# Autodesk Inventor assembly: 21-091-PHANTOM-HRDSET
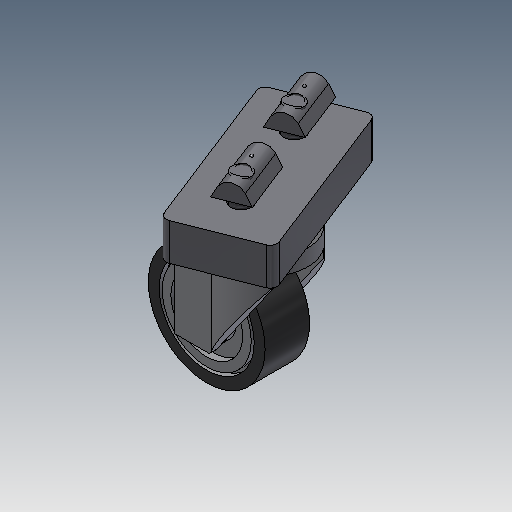
[picture p0: Inventor's stored thumbnail of the model, 512x512]
Saved by Autodesk Inventor 2018.3 (Build 223284000, 284)
## iProperties
Created: 2004-11-19
Part Number: 21-091-PHANTOM-HRDSET
Document SubType Name: Assembly
Designer: Autodesk, Inc.
Manufacturer: Standard
Standards Organization: Custom
Description: PHANTOM, CASTER, HARDWARE SET
Catalog Web Link: http://www.parker.com/ead/cm1.asp?cmid=809
Vendor: PARKER IPS
Mass: 438.641 g
Surface Area: 350.867 cm^2
Volume: 101.464 cm^3
Density: 4.3231 g/cm^3
CAGE: 1LJX3
Dept. ID: Product Design
Description #2: ---
Finish #1: ---
Finish #2: ---
Material ID: ---
Project Number: ---
Author: Autodesk, Inc.
## Documents named in this file (4)
- C:\AVAInvAPI\Workspace\Test Station\Components\21-091 Caster Phantom.iam
- C:\AVAInvAPI\Workspace\Test Station\Components\21-091 Caster.ipt
- C:\AVAInvAPI\Workspace\Test Station\Components\21-09x_Caster_Mnt_Phantom.iam
- C:\AVAInvAPI\Workspace\Test Station\Components\M10x25-Spring Phantom.iam
## Components (3 placed, 3 different names)
1. 21-091 Caster:1
2. 21-09x_Caster_Mnt_Phantom:1 [sub-assembly]
3. M10x25-Spring Phantom:1 [sub-assembly]
## Relationships (2: Insert 2)
- [Insert]: 21-091 Caster:1 ↔ M10x25-Spring Phantom:1
- [Insert]: 21-091 Caster:1 ↔ 21-09x_Caster_Mnt_Phantom:1
